# Autodesk Inventor assembly: BoltWasher4x10
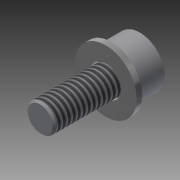
[picture p0: Inventor's stored thumbnail of the model, 180x180]
Saved by Autodesk Inventor 2016 (Build 200138000, 138)
## iProperties
Category: Hardware
Created: 2015-01-27
Part Number: BoltWasher4x10
Document SubType Name: Assembly
Designer: Jack
Vendor: McMaster Carr
Mass: 0.54014 g
Surface Area: 4.44453 cm^2
Volume: 0.288561 cm^3
Density: 1.87184 g/cm^3
Author: Jack
Title: Bolt + Washer 3x24
## Documents named in this file (3)
- C:\Users\Jack\ownCloud\Projects\CrossBot\InventorModel\Hardware\BoltWashers\BoltWasher4\BoltWasher4x10.iam
- C:\Users\Jack\ownCloud\Projects\CrossBot\InventorModel\Hardware\Wahsers\M4Washer.ipt
- C:\Users\Jack\ownCloud\Projects\CrossBot\InventorModel\Hardware\Bolts\SHCS\SHCS4\SHCS4x10.ipt
## Components (2 placed, 2 different names)
1. M4Washer:1 — Mate:1, Mate:2
2. SHCS4x10:1 — Mate:1, Mate:2
## Relationships (2: Mate 2)
- Mate:1: M4Washer:1 ↔ SHCS4x10:1
- Mate:2: M4Washer:1 ↔ SHCS4x10:1
